# Autodesk Inventor assembly: Assembly_NV_Module
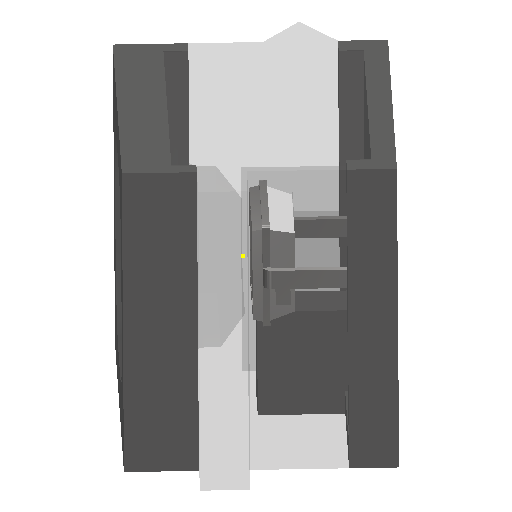
[picture p0: Inventor's stored thumbnail of the model, 512x512]
Saved by Autodesk Inventor 2026.1 (Build 301233020, 233B)
## iProperties
Created: 2026-01-26
Part Number: Assembly_NV_Module
Document SubType Name: Assembly
Designer: samuel
Author: samuel
## Documents named in this file (6)
- E:\Fraunhofer\Design\Assembly_NV_Module.iam
- E:\Fraunhofer\Design\Optical module_lid.ipt
- E:\Fraunhofer\Design\NV_module.ipt
- E:\Fraunhofer\Design\NV_module_lid_2.ipt
- E:\Fraunhofer\Design\Parts\nv_FILTER.ipt
- E:\Fraunhofer\Design\Parts\bpw34\bpw34\bpw34.iam
## Components (5 placed, 5 different names)
1. Optical module_lid:1 — Flush:5, Flush:6, Mate:10
2. NV_module:1 — Mate:5, Mate:6, Mate:7, Flush:3, Flush:4, Mate:8, Flush:5, Flush:6, Mate:9, Mate:10
3. NV_module_lid_2:1 — Flush:3, Flush:4, Mate:9
4. nv_FILTER:1 — Mate:8
5. bpw34:1 [sub-assembly] — Mate:5, Mate:6, Mate:7
## Relationships (10: Mate 6, Flush 4)
- Mate:5: NV_module:1 ↔ bpw34:1
- Mate:6: NV_module:1 ↔ bpw34:1
- Mate:7 (1.5 mm): NV_module:1 ↔ bpw34:1
- Flush:3: NV_module:1 ↔ NV_module_lid_2:1
- Flush:4: NV_module:1 ↔ NV_module_lid_2:1
- Mate:8: NV_module:1 ↔ nv_FILTER:1
- Flush:5: Optical module_lid:1 ↔ NV_module:1
- Flush:6: Optical module_lid:1 ↔ NV_module:1
- Mate:9: NV_module:1 ↔ NV_module_lid_2:1
- Mate:10: Optical module_lid:1 ↔ NV_module:1
